# Autodesk Inventor assembly: Lumbar
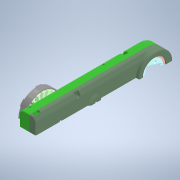
[picture p0: Inventor's stored thumbnail of the model, 180x180]
Saved by Autodesk Inventor 2022.2 (Build 262287000, 287)
## iProperties
Created: 2022-01-12
Part Number: Lumbar
Document SubType Name: Assembly
Designer: Jochen
Author: Jochen
## Documents named in this file (7)
- D:\Projects\Chewbacca\CAD\Lumbar\Lumbar.iam
- D:\Projects\Chewbacca\CAD\Lumbar\Lumbar.ipt
- D:\Projects\Chewbacca\CAD\Common\Motor\MotorModule.iam
- D:\Projects\Chewbacca\CAD\Common\Motor\TransmissionPuileyCenter.iam
- D:\Projects\Chewbacca\CAD\Common\Motor\Transmission Pulley.iam
- D:\Projects\Chewbacca\CAD\Common\Belt Tensioner\BeltTensioner 10mm.iam
- D:\Projects\Chewbacca\CAD\Common\Belt Tensioner\MotorBeltTensioner 10mm.iam
## Components (6 placed, 6 different names)
1. Lumbar:1 — Mate:1, Mate:2, Mate:3, Mate:4, Mate:5, Mate:6, Mate:7, Mate:8, Mate:9, Mate:10
2. MotorModule:1 [sub-assembly] — Mate:1, Mate:2
3. TransmissionPuileyCenter:1 [sub-assembly] — Mate:3, Mate:4
4. Transmission Pulley:1 [sub-assembly] — Mate:5, Mate:6
5. Belt tensioner 10mm:1 [sub-assembly] — Mate:7, Mate:8
6. MotorBeltTensioner 10mm:1 [sub-assembly] — Mate:9, Mate:10
## Relationships (10: Mate 10)
- Mate:1: Lumbar:1 ↔ MotorModule:1
- Mate:2: Lumbar:1 ↔ MotorModule:1
- Mate:3: Lumbar:1 ↔ TransmissionPuileyCenter:1
- Mate:4: Lumbar:1 ↔ TransmissionPuileyCenter:1
- Mate:5: Lumbar:1 ↔ Transmission Pulley:1
- Mate:6: Lumbar:1 ↔ Transmission Pulley:1
- Mate:7: Lumbar:1 ↔ Belt tensioner 10mm:1
- Mate:8: Lumbar:1 ↔ Belt tensioner 10mm:1
- Mate:9: Lumbar:1 ↔ MotorBeltTensioner 10mm:1
- Mate:10: Lumbar:1 ↔ MotorBeltTensioner 10mm:1
